# Autodesk Inventor assembly: Absauganlage
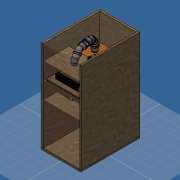
[picture p0: Inventor's stored thumbnail of the model, 180x180]
Saved by Autodesk Inventor 2019 (Build 230136000, 136)
## iProperties
Created: 2020-08-02
Part Number: Absauganlage
Material: Generisch
Document SubType Name: Assembly
Designer: Stefan
Mass: 54680.4 g
Surface Area: 87708.3 cm^2
Volume: 54603.6 cm^3
Density: 1.00141 g/cm^3
Author: Stefan
## Documents named in this file (8)
- C:\Users\User\OneDrive\Dokumente\Inventor\Absauganlage\Absauganlage.iam
- C:\Users\User\OneDrive\Dokumente\Inventor\Absauganlage\Korpus.iam
- C:\Users\User\OneDrive\Dokumente\Inventor\Absauganlage\Zyklon.iam
- C:\Users\User\OneDrive\Dokumente\Inventor\Absauganlage\Korpus_Einbau.iam
- C:\Users\User\OneDrive\Dokumente\Inventor\Absauganlage\Front_Staubfach.ipt
- C:\Users\User\OneDrive\Dokumente\Inventor\Absauganlage\Front_Fach.ipt
- C:\Users\User\OneDrive\Dokumente\Inventor\Absauganlage\Front_Elektronik.ipt
- C:\Users\User\OneDrive\Dokumente\Inventor\Absauganlage\Import\HT_Rohr\HT-50-45°-3-66.iam
## Components (15 placed, 7 different names)
1. Korpus:1 [sub-assembly] — Passend:1, Fluchtend:1, Winkel:1, Passend:2, Passend:3, Fluchtend:2, Passend:4, Passend:5, Passend:6, Passend:7, Passend:9, Passend:10, Passend:11, Passend:14
2. Zyklon:1 [sub-assembly] — Passend:1, Fluchtend:1, Winkel:1, Passend:18, Passend:19, Passend:32
3. Korpus_Einbau:1 [sub-assembly] — Passend:2, Passend:3, Fluchtend:2, Passend:8, Passend:12, Passend:13, Passend:15, Passend:22, Fluchtend:7
4. Front_Staubfach:1 — Passend:4, Passend:5, Passend:11
5. Front_Fach:1 — Passend:8, Passend:9, Passend:12
6. Front_Fach:2 — Passend:6, Passend:7, Passend:10
7. Front_Elektronik:1 — Passend:13, Passend:14, Passend:15, Winkel:2
8. HT-50-45°-3-66:1 [sub-assembly] — Passend:16, Passend:17, Fluchtend:3, Passend:18, Passend:19
9. HT-50-45°-3-66:2 [sub-assembly] — Passend:16, Passend:17, Fluchtend:3, Passend:23
10. HT-50-45°-3-66:3 [sub-assembly] — Passend:20, Passend:21, Fluchtend:4, Passend:22
11. HT-50-45°-3-66:4 [sub-assembly] — Passend:20, Passend:21, Fluchtend:4, Passend:23
12. HT-50-45°-3-66:6 [sub-assembly] — Passend:24, Passend:25, Passend:32
13. HT-50-45°-3-66:5 [sub-assembly] — Passend:24, Passend:25, Passend:30
14. HT-50-45°-3-66:8 [sub-assembly] — Passend:28, Passend:29, Fluchtend:6, Passend:30
15. HT-50-45°-3-66:7 [sub-assembly] — Passend:28, Passend:29, Fluchtend:6, Fluchtend:8, Winkel:2
## Relationships (38: Mate 29, Flush 7, Angle 2)
- Passend:1 [Mate]: Korpus:1 ↔ Zyklon:1
- Fluchtend:1 [Flush] (200 mm): Korpus:1 ↔ Zyklon:1
- Winkel:1 [Angle] (40 deg): Korpus:1 ↔ Zyklon:1
- Passend:2 [Mate]: Korpus:1 ↔ Korpus_Einbau:1
- Passend:3 [Mate]: Korpus:1 ↔ Korpus_Einbau:1
- Fluchtend:2 [Flush]: Korpus:1 ↔ Korpus_Einbau:1
- Passend:4 [Mate]: Korpus:1 ↔ Front_Staubfach:1
- Passend:5 [Mate]: Korpus:1 ↔ Front_Staubfach:1
- Passend:6 [Mate]: Korpus:1 ↔ Front_Fach:2
- Passend:7 [Mate]: Korpus:1 ↔ Front_Fach:2
- Passend:8 [Mate]: Korpus_Einbau:1 ↔ Front_Fach:1
- Passend:9 [Mate]: Korpus:1 ↔ Front_Fach:1
- Passend:10 [Mate]: Korpus:1 ↔ Front_Fach:2
- Passend:11 [Mate]: Korpus:1 ↔ Front_Staubfach:1
- Passend:12 [Mate]: Korpus_Einbau:1 ↔ Front_Fach:1
- Passend:13 [Mate]: Korpus_Einbau:1 ↔ Front_Elektronik:1
- Passend:14 [Mate]: Korpus:1 ↔ Front_Elektronik:1
- Passend:15 [Mate]: Korpus_Einbau:1 ↔ Front_Elektronik:1
- Passend:16 [Mate]: HT-50-45°-3-66:1 ↔ HT-50-45°-3-66:2
- Passend:17 [Mate]: HT-50-45°-3-66:1 ↔ HT-50-45°-3-66:2
- Fluchtend:3 [Flush]: HT-50-45°-3-66:1 ↔ HT-50-45°-3-66:2
- Passend:18 [Mate]: Zyklon:1 ↔ HT-50-45°-3-66:1
- Passend:19 [Mate]: Zyklon:1 ↔ HT-50-45°-3-66:1
- Passend:20 [Mate]: HT-50-45°-3-66:3 ↔ HT-50-45°-3-66:4
- Passend:21 [Mate]: HT-50-45°-3-66:3 ↔ HT-50-45°-3-66:4
- Fluchtend:4 [Flush]: HT-50-45°-3-66:3 ↔ HT-50-45°-3-66:4
- Passend:22 [Mate]: Korpus_Einbau:1 ↔ HT-50-45°-3-66:3
- Passend:23 [Mate]: HT-50-45°-3-66:2 ↔ HT-50-45°-3-66:4
- Passend:24 [Mate]: HT-50-45°-3-66:6 ↔ HT-50-45°-3-66:5
- Passend:25 [Mate]: HT-50-45°-3-66:6 ↔ HT-50-45°-3-66:5
- Passend:28 [Mate]: HT-50-45°-3-66:8 ↔ HT-50-45°-3-66:7
- Passend:29 [Mate]: HT-50-45°-3-66:8 ↔ HT-50-45°-3-66:7
- Fluchtend:6 [Flush]: HT-50-45°-3-66:8 ↔ HT-50-45°-3-66:7
- Passend:30 [Mate]: HT-50-45°-3-66:5 ↔ HT-50-45°-3-66:8
- Fluchtend:7 [Flush] (-60 mm): Korpus_Einbau:1
- Fluchtend:8 [Flush]: HT-50-45°-3-66:7
- Passend:32 [Mate]: Zyklon:1 ↔ HT-50-45°-3-66:6
- Winkel:2 [Angle] (0 deg): Front_Elektronik:1 ↔ HT-50-45°-3-66:7
